# Autodesk Inventor assembly: UltrasonicSensor2
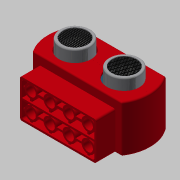
[picture p0: Inventor's stored thumbnail of the model, 180x180]
Saved by Autodesk Inventor 2019.3 (Build 233278000, 278)
## iProperties
Created: 2019-02-04
Part Number: UltrasonicSensor2
Document SubType Name: Assembly
Designer: Varga Daniel
Sending System: SolidWorks 2018
Last Author: david
Last Saved: 2019-02-07
Author: Varga Daniel
## Documents named in this file (5)
- C:\!_Dani\!_cloud\OneDrive\!_munka\Revolution\RevvyDemoKit\Structural parts\Demo parts\Ultrasonic sensor\Inventor imported\UltrasonicSensor2.iam
- C:\!_Dani\!_cloud\OneDrive\!_munka\Revolution\RevvyDemoKit\Structural parts\Demo parts\Ultrasonic sensor\Inventor imported\HC-SR04.ipt
- C:\!_Dani\!_cloud\OneDrive\!_munka\Revolution\RevvyDemoKit\Structural parts\Demo parts\Ultrasonic sensor\Inventor imported\rj45_vert.ipt
- C:\!_Dani\!_cloud\OneDrive\!_munka\Revolution\RevvyDemoKit\Structural parts\Demo parts\Ultrasonic sensor\Inventor imported\UScA_1.ipt
- C:\!_Dani\!_cloud\OneDrive\!_munka\Revolution\RevvyDemoKit\Structural parts\Demo parts\Ultrasonic sensor\Inventor imported\UScA_2.ipt
## Components (4 placed, 4 different names)
1. HC-SR04:1 — Mate:1, Mate:3
2. rj45_vert:1 — Mate:2, Flush:2
3. UScA_1:1 — Mate:1, Mate:2, Flush:1, Flush:2, Mate:4
4. UScA_2:1 — Mate:3, Flush:1, Mate:4
## Relationships (6: Mate 4, Flush 2)
- Mate:1: HC-SR04:1 ↔ UScA_1:1
- Mate:2: rj45_vert:1 ↔ UScA_1:1
- Mate:3: HC-SR04:1 ↔ UScA_2:1
- Flush:1: UScA_1:1 ↔ UScA_2:1
- Flush:2: rj45_vert:1 ↔ UScA_1:1
- Mate:4: UScA_1:1 ↔ UScA_2:1
